# Autodesk Inventor assembly: talon plate subassy
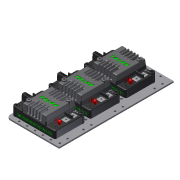
[picture p0: Inventor's stored thumbnail of the model, 180x180]
Saved by Autodesk Inventor 2015 (Build 190159000, 159)
## iProperties
Created: 2015-02-10
Part Number: talon plate subassy
Document SubType Name: Assembly
Designer: sspriggs
Mass: 157.834 g
Surface Area: 1475.55 cm^2
Volume: 157.834 cm^3
Density: 1 g/cm^3
Author: sspriggs
## Documents named in this file (3)
- H:\2015\Workspaces\Workspace\electronics parts\talon plate subassy.iam
- H:\2015\Workspaces\Workspace\electronics parts\talon plate.ipt
- H:\2015\Workspaces\Workspace\electronics parts\Talon.ipt
## Components (4 placed, 2 different names)
1. talon plate:1 — Flush:5
2. Talon:1 — Flush:1, Flush:2, Flush:3, Flush:4, Flush:5
3. Talon:2 — Flush:1, Flush:3
4. Talon:3 — Flush:2, Flush:4
## Relationships (5: Flush 5)
- Flush:1: Talon:1 ↔ Talon:2
- Flush:2: Talon:1 ↔ Talon:3
- Flush:3: Talon:1 ↔ Talon:2
- Flush:4: Talon:1 ↔ Talon:3
- Flush:5: talon plate:1 ↔ Talon:1
